# Autodesk Inventor assembly: Ensamblaje carcasa control
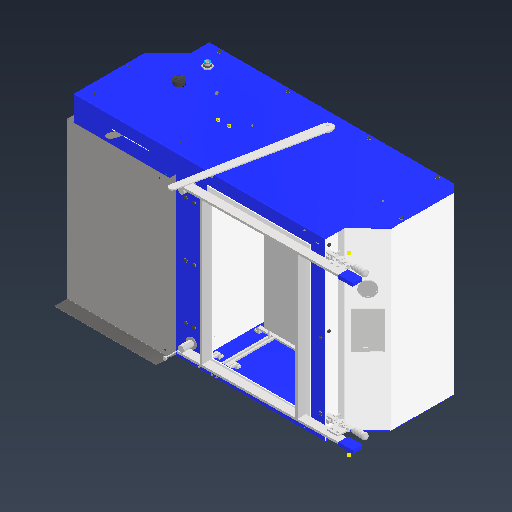
[picture p0: Inventor's stored thumbnail of the model, 512x512]
Saved by Autodesk Inventor 2021 (Build 250183000, 183)
## iProperties
Created: 2021-04-15
Part Number: Ensamblaje carcasa control
Document SubType Name: Assembly
Designer: Admin
Author: Admin
## Documents named in this file (40)
- J:\PAI\Proyecto_PAI_2021\01 CAD\Ensamblaje carcasa control.iam
- J:\PAI\Proyecto_PAI_2021\01 CAD\Carcasa_azul.ipt
- J:\PAI\Proyecto_PAI_2021\01 CAD\Carcaza_blanca_frontal.ipt
- J:\PAI\Proyecto_PAI_2021\01 CAD\Tapa_blanca_inferior.ipt
- J:\PAI\Proyecto_PAI_2021\01 CAD\Vacuometro.ipt
- J:\PAI\Proyecto_PAI_2021\01 CAD\HMI_NV3W_MR20L_V1.iam
- J:\PAI\Proyecto_PAI_2021\01 CAD\Receptaculo e interruptor.ipt
- J:\PAI\Proyecto_PAI_2021\01 CAD\Portafusible para fusible de 13A.ipt
- J:\PAI\Proyecto_PAI_2021\01 CAD\Tapa_interior_1.ipt
- J:\PAI\Proyecto_PAI_2021\01 CAD\Tapa_interior_2.ipt
- J:\PAI\Proyecto_PAI_2021\01 CAD\Tapa_blanca_trasera.ipt
- J:\PAI\Proyecto_PAI_2021\01 CAD\Bomba de Vacio.ipt
- J:\PAI\Proyecto_PAI_2021\01 CAD\Marco molde.ipt
- J:\PAI\Proyecto_PAI_2021\01 CAD\CSN 02 1721 - 17,5.ipt
- J:\PAI\Proyecto_PAI_2021\01 CAD\Ensamblaje_soportme molde_barras.iam
- J:\PAI\Proyecto_PAI_2021\01 CAD\Mecanismo Modelado.iam
- J:\PAI\Proyecto_PAI_2021\01 CAD\Bandeja_proteccion_carcasa_control.ipt
- J:\PAI\Proyecto_PAI_2021\01 CAD\BS 4320 - M5 (Forma A).ipt
- J:\PAI\Proyecto_PAI_2021\01 CAD\ISO 7380-1 - M5 x 8.ipt
- J:\PAI\Proyecto_PAI_2021\01 CAD\BS 4183 - M5(1).ipt
- J:\PAI\Proyecto_PAI_2021\01 CAD\MecanismoBoqueoCarro\ProtectorBloqueo.ipt
- J:\PAI\Proyecto_PAI_2021\01 CAD\Ensamble eléctrico.iam
- J:\PAI\Proyecto_PAI_2021\01 CAD\ISO 7049 - ST 3,5 x 9,5 - C - H.ipt
- J:\PAI\Proyecto_PAI_2021\01 CAD\020sa24.iam
- J:\PAI\Proyecto_PAI_2021\01 CAD\ls-s02-zb.iam
- J:\PAI\Proyecto_PAI_2021\01 CAD\Racor bomba.ipt
- J:\PAI\Proyecto_PAI_2021\01 CAD\2021 C-1_8-P-6.ipt
- J:\PAI\Proyecto_PAI_2021\01 CAD\153160 QSS-10.iam
- J:\PAI\Proyecto_PAI_2021\01 CAD\15631 N-1_4-P-6-MS.ipt
- J:\PAI\Proyecto_PAI_2021\01 CAD\Filtro.iam
- J:\PAI\Proyecto_PAI_2021\01 CAD\Base vacuometro.ipt
- J:\PAI\Proyecto_PAI_2021\01 CAD\BS 4168 - M4 x 20(1).ipt
- J:\PAI\Proyecto_PAI_2021\01 CAD\AS 1112 - M4(2).ipt
- C:\Users\GABRIEL LOL\Desktop\planos pai\mecanismobloq2\MecanismoBloq2.iam
- C:\Users\GABRIEL LOL\Desktop\planos pai\PieDeBomba.iam
- C:\Users\GABRIEL LOL\Documents\Inventor\Content Center Files\R2021\en-US\ISO 7380-1\ISO 7380-1 - M6 x 16.ipt
- C:\Users\GABRIEL LOL\Documents\Inventor\Content Center Files\R2021\en-US\ISO 7092\ISO 7092 - ST 2.5 - 140 HV.ipt
- C:\Users\GABRIEL LOL\Documents\Inventor\Content Center Files\R2021\en-US\ISO 4762(2)\ISO 4762 - M2.5 x 10ISO.ipt
- C:\Users\GABRIEL LOL\Documents\Inventor\Content Center Files\R2021\en-US\ISO 4032(2)\ISO 4032 - M2.5 - ISO.ipt
- C:\Users\GABRIEL LOL\Documents\Inventor\Content Center Files\R2021\en-US\ISO 4762(2)\ISO 4762 - M2.5 x 8ISO.ipt
## Components (183 placed, 39 different names)
1. Carcasa_azul:1 — Coincidencia:1, Nivelación:1, Coincidencia:2, Coincidencia:3, Nivelación:2, Coincidencia:5, Coincidencia:6, Coincidencia:7, Coincidencia:8, Coincidencia:9, Coincidencia:18, Coincidencia:20, Coincidencia:27, Nivelación:6, Nivelación:7, Coincidencia:28, Coincidencia:29, Coincidencia:30, Coincidencia:31, Coincidencia:32, Coincidencia:34, Nivelación:8, Nivelación:9, Coincidencia:35, De rotación:1, De rotación:2, De rotación:4, De rotación:5, De rotación:6, De rotación:7, De rotación:8, De rotación:9, De rotación:10, De rotación:11, De rotación:42, De rotación:48, De rotación:64, De rotación:65, De rotación:66, Coincidencia:36, Mate:38, Coincidencia:39, De rotación:107, De rotación:108, De rotación:109, De rotación:110, De rotación:111, De rotación:112, De rotación:117, Mate:40, Mate:41, Mate:42, Coincidencia:45, Coincidencia:46, De rotación:118, De rotación:119, De rotación:120, De rotación:121, De rotación:122, De rotación:123, Mate:71, Mate:72, Mate:80, Mate:102, Mate:103, Mate:104, Mate:106, Mate:107, Mate:108, Mate:110, Mate:111, Mate:112, Mate:114, Mate:115, Mate:116, Mate:118, Mate:119, Mate:120, Mate:122, Mate:123, Mate:124, Mate:126, Mate:127, Mate:128, Mate:129, Mate:130, Mate:132, Mate:134, Mate:135, Mate:136, Mate:138, Mate:139, Mate:140, Mate:141, Mate:142, Mate:144
2. Carcaza_blanca_frontal:1 — Coincidencia:1, Nivelación:1, Coincidencia:2, Coincidencia:4, Coincidencia:10, Coincidencia:11, Coincidencia:12, Coincidencia:13, Coincidencia:14, Coincidencia:19, De rotación:24, De rotación:25, De rotación:26, De rotación:56, De rotación:57, De rotación:58, Coincidencia:77
3. Tapa_blanca_inferior:1 — Coincidencia:3, Coincidencia:4, Nivelación:2, Nivelación:4, Coincidencia:21, De rotación:38, De rotación:39, De rotación:40, De rotación:41, De rotación:44, De rotación:45, De rotación:46, De rotación:49, De rotación:50, De rotación:51, De rotación:52, De rotación:98, De rotación:99, De rotación:100, De rotación:124, De rotación:125, De rotación:126, De rotación:127, De rotación:128, De rotación:129, Mate:49, Mate:81, Mate:82, Mate:83, Mate:84, Mate:85, Mate:86, Mate:87, Mate:88, Mate:101, Insert:1, Insert:2, Insert:3, Insert:4
4. Vacuometro:1 — Coincidencia:10, Coincidencia:11, Mate:69, Mate:70, Coincidencia:78, Coincidencia:79, De rotación:142, De rotación:143
5. HMI_NV3W_MR20L_V1:1 [sub-assembly] — Coincidencia:12, Coincidencia:13, Coincidencia:14
6. Receptaculo e interruptor:1 — Coincidencia:7, Coincidencia:8, Coincidencia:9
7. Portafusible para fusible de 13A:1 — Coincidencia:5, Coincidencia:6
8. Tapa_interior_2:1 — Coincidencia:18, Coincidencia:19, De rotación:62, De rotación:63, Rígido:1, Coincidencia:44
9. Tapa_blanca_trasera:1 — Coincidencia:20, Nivelación:4, Coincidencia:21, De rotación:104, De rotación:105, De rotación:106
10. Marco molde:1 — Coincidencia:27, Nivelación:6, Nivelación:7
11. CSN 02 1721 17,5:1 — Coincidencia:28, Coincidencia:30, Cilíndrica:1
12. CSN 02 1721 17,5:2 — Coincidencia:29, Coincidencia:31
13. Ensamblaje_soportme molde_barras:1 [sub-assembly] — Cilíndrica:1
14. Mecanismo Modelado:1 [sub-assembly] — Coincidencia:32, Coincidencia:34, Coincidencia:36, Mate:37, Mate:105, Mate:109, Mate:113, Mate:117, Mate:121, Mate:125, Mate:131, Mate:133, Mate:137, Mate:143, Mate:145
15. Bandeja_proteccion_carcasa_control:1 — Nivelación:8, Nivelación:9, Coincidencia:35
16. BS 4320 Forma AB M5 (Forma A):4 — De rotación:1, De rotación:16
17. BS 4320 Forma AB M5 (Forma A):5 — De rotación:2, De rotación:15
18. BS 4320 Forma AB M5 (Forma A):7 — De rotación:4, De rotación:14
19. BS 4320 Forma AB M5 (Forma A):8 — De rotación:5, De rotación:17
20. BS 4320 Forma AB M5 (Forma A):9 — De rotación:6, De rotación:13
21. BS 4320 Forma AB M5 (Forma A):10 — De rotación:9, De rotación:21
22. BS 4320 Forma AB M5 (Forma A):11 — De rotación:7, De rotación:23
23. BS 4320 Forma AB M5 (Forma A):12 — De rotación:11, De rotación:19
24. BS 4320 Forma AB M5 (Forma A):13 — De rotación:8, De rotación:22
25. BS 4320 Forma AB M5 (Forma A):14 — De rotación:10, De rotación:20
26. ISO 7380-1 M5 x 8:1 — De rotación:15
27. ISO 7380-1 M5 x 8:3 — De rotación:17
28. ISO 7380-1 M5 x 8:4 — De rotación:16
29. ISO 7380-1 M5 x 8:5 — De rotación:14
30. ISO 7380-1 M5 x 8:6 — De rotación:13
31. ISO 7380-1 M5 x 8:7 — De rotación:20
32. ISO 7380-1 M5 x 8:8 — De rotación:21
33. ISO 7380-1 M5 x 8:10 — De rotación:23
34. ISO 7380-1 M5 x 8:11 — De rotación:19
35. ISO 7380-1 M5 x 8:12 — De rotación:22
36. ISO 7380-1 M5 x 8:13 — De rotación:27
37. ISO 7380-1 M5 x 8:14 — De rotación:29
38. ISO 7380-1 M5 x 8:15 — De rotación:28
39. BS 4320 Forma AB M5 (Forma A):16 — De rotación:26, De rotación:27
40. BS 4320 Forma AB M5 (Forma A):17 — De rotación:25, De rotación:28
41. BS 4320 Forma AB M5 (Forma A):18 — De rotación:24, De rotación:29
42. BS 4183 - Métrico M5:1 — De rotación:38
43. BS 4183 - Métrico M5:2 — De rotación:39
44. BS 4183 - Métrico M5:3 — De rotación:42
45. BS 4183 - Métrico M5:4 — De rotación:40
46. BS 4183 - Métrico M5:6 — De rotación:41
47. BS 4183 - Métrico M5:7 — De rotación:45
48. BS 4183 - Métrico M5:8 — De rotación:44
49. BS 4183 - Métrico M5:10 — De rotación:46
50. BS 4183 - Métrico M5:11 — De rotación:48
51. BS 4183 - Métrico M5:12 — De rotación:49
52. BS 4183 - Métrico M5:13 — De rotación:50
53. BS 4183 - Métrico M5:14 — De rotación:52
54. BS 4183 - Métrico M5:15 — De rotación:51
55. ISO 7380-1 M5 x 8:21 — De rotación:59
56. ISO 7380-1 M5 x 8:22 — De rotación:60
57. ISO 7380-1 M5 x 8:23 — De rotación:61
58. BS 4320 Forma AB M5 (Forma A):22 — De rotación:57, De rotación:60
59. BS 4320 Forma AB M5 (Forma A):23 — De rotación:58, De rotación:61
60. BS 4320 Forma AB M5 (Forma A):24 — De rotación:56, De rotación:59
61. BS 4183 - Métrico M5:19 — De rotación:62
62. BS 4183 - Métrico M5:20 — De rotación:63
63. BS 4183 - Métrico M5:21 — Rígido:1
64. ISO 7380-1 M5 x 8:24 — De rotación:69
65. ISO 7380-1 M5 x 8:25 — De rotación:68
66. ISO 7380-1 M5 x 8:26 — De rotación:67
67. BS 4320 Forma AB M5 (Forma A):25 — De rotación:66, De rotación:69
68. BS 4320 Forma AB M5 (Forma A):26 — De rotación:65, De rotación:68
69. BS 4320 Forma AB M5 (Forma A):27 — De rotación:64, De rotación:67
70. BS 4183 - Métrico M5:22
71. BS 4183 - Métrico M5:23
72. BS 4183 - Métrico M5:24
73. ProtectorBloqueo:1 — Mate:37, Mate:38
74. Tapa_interior_1:1 — Coincidencia:39, Coincidencia:44, Coincidencia:47
75. Ensamble eléctrico:1 [sub-assembly] — Coincidencia:45, Coincidencia:46, Coincidencia:47, De rotación:146, De rotación:147, De rotación:148, De rotación:149
76. ISO 7380-1 M5 x 8:39 — De rotación:101
77. ISO 7380-1 M5 x 8:40 — De rotación:102
78. ISO 7380-1 M5 x 8:41 — De rotación:103
79. BS 4320 Forma AB M5 (Forma A):40 — De rotación:98, De rotación:101
80. BS 4320 Forma AB M5 (Forma A):41 — De rotación:99, De rotación:102
81. BS 4320 Forma AB M5 (Forma A):42 — De rotación:100, De rotación:103
82. ISO 7049 - C-H ST 3,5 x 9,5 - C - H:1 — De rotación:106
83. ISO 7049 - C-H ST 3,5 x 9,5 - C - H:2 — De rotación:105
84. ISO 7049 - C-H ST 3,5 x 9,5 - C - H:3 — De rotación:104
85. ISO 7049 - C-H ST 3,5 x 9,5 - C - H:4 — De rotación:108
86. ISO 7049 - C-H ST 3,5 x 9,5 - C - H:5 — De rotación:107
87. BS 4320 Forma AB M5 (Forma A):43 — De rotación:112, De rotación:115
88. BS 4320 Forma AB M5 (Forma A):44 — De rotación:111, De rotación:116
89. BS 4320 Forma AB M5 (Forma A):45 — De rotación:110, De rotación:114
90. BS 4320 Forma AB M5 (Forma A):46 — De rotación:109, De rotación:113
91. ISO 7380-1 M5 x 8:42 — De rotación:114
92. ISO 7380-1 M5 x 8:43 — De rotación:113
93. ISO 7380-1 M5 x 8:44 — De rotación:116
94. ISO 7380-1 M5 x 8:45 — De rotación:115
95. BS 4183 - Métrico M5:25 — De rotación:117
96. 020sa24:1 [sub-assembly] — Mate:40, Mate:41
97. ls-s02-zb:1 [sub-assembly] — Mate:42
98. BS 4320 Forma AB M5 (Forma A):47 — De rotación:120, De rotación:133
99. BS 4320 Forma AB M5 (Forma A):48 — De rotación:123, De rotación:130
100. BS 4320 Forma AB M5 (Forma A):49 — De rotación:121, De rotación:132
101. BS 4320 Forma AB M5 (Forma A):50 — De rotación:122, De rotación:131
102. BS 4320 Forma AB M5 (Forma A):51 — De rotación:119, De rotación:134
103. BS 4320 Forma AB M5 (Forma A):52 — De rotación:118, De rotación:135
104. BS 4320 Forma AB M5 (Forma A):53 — De rotación:125, De rotación:141
105. BS 4320 Forma AB M5 (Forma A):54 — De rotación:127, De rotación:139
106. BS 4320 Forma AB M5 (Forma A):55 — De rotación:128, De rotación:136
107. BS 4320 Forma AB M5 (Forma A):56 — De rotación:129, De rotación:137
108. BS 4320 Forma AB M5 (Forma A):57 — De rotación:126, De rotación:138
109. BS 4320 Forma AB M5 (Forma A):58 — De rotación:124, De rotación:140
110. ISO 7380-1 M5 x 8:46 — De rotación:130
111. ISO 7380-1 M5 x 8:47 — De rotación:132
112. ISO 7380-1 M5 x 8:48 — De rotación:135
113. ISO 7380-1 M5 x 8:49 — De rotación:134
114. ISO 7380-1 M5 x 8:50 — De rotación:131
115. ISO 7380-1 M5 x 8:51 — De rotación:133
116. ISO 7380-1 M5 x 8:52 — De rotación:136
117. ISO 7380-1 M5 x 8:53 — De rotación:137
118. ISO 7380-1 M5 x 8:54 — De rotación:138
119. ISO 7380-1 M5 x 8:55 — De rotación:139
120. ISO 7380-1 M5 x 8:56 — De rotación:141
121. ISO 7380-1 M5 x 8:57 — De rotación:140
122. Bomba de Vacio:1 — Mate:49, Mate:50, Mate:51, Mate:52, Mate:53, Mate:89, Mate:90, Mate:91, Mate:92, Mate:93, Mate:94, Mate:95, Mate:96, Mate:97, Mate:98, Mate:99
123. Racor bomba:1 — Mate:50, Mate:51
124. Racor bomba:2 — Mate:52, Mate:53
125. Racor bomba:3 — De rotación:146
126. Racor bomba:4 — De rotación:147
127. Racor bomba:5 — De rotación:149
128. 2021 C-1_8-P-6:1 — Mate:69, Mate:70
129. 153160 QSS-10:1 [sub-assembly] — Mate:71, Mate:72
130. 15631 N-1_4-P-6-MS:2 — De rotación:148
131. Filtro:1 [sub-assembly]
132. Base vacuometro:1 — Coincidencia:77, Coincidencia:78, Coincidencia:79, De rotación:144, De rotación:145
133. BS 4168 : Pieza 1 Tornillo de cabeza cilíndrica con hueco hexagonal - Métrico M4 x 20:1 — De rotación:143
134. BS 4168 : Pieza 1 Tornillo de cabeza cilíndrica con hueco hexagonal - Métrico M4 x 20:2 — De rotación:142
135. AS 1112 (4) - Métrico M4:1 — De rotación:144
136. AS 1112 (4) - Métrico M4:2 — De rotación:145
137. MecanismoBloq2:1 [sub-assembly] — Mate:80
138. PieDeBomba:1 [sub-assembly] — Mate:81, Mate:85, Mate:89, Mate:91, Mate:100
139. PieDeBomba:2 [sub-assembly] — Mate:84, Mate:87
140. PieDeBomba:3 [sub-assembly] — Mate:83, Mate:88, Mate:90
141. PieDeBomba:4 [sub-assembly] — Mate:82, Mate:86
142. ISO 7380-1 M6 x 16:1 — Mate:92, Mate:93
143. ISO 7380-1 M6 x 16:2 — Mate:94, Mate:95
144. ISO 7380-1 M6 x 16:3 — Mate:96, Mate:97
145. ISO 7380-1 M6 x 16:4 — Mate:98, Mate:99
146. ISO 7380-1 M6 x 16:5 — Mate:100, Mate:101
147. ISO 7380-1 M6 x 16:6 — Insert:1
148. ISO 7380-1 M6 x 16:7 — Insert:2
149. ISO 7380-1 M6 x 16:8 — Insert:3
150. ISO 7380-1 M6 x 16:9 — Insert:4
151. ISO 7092 ST 2.5 - 140 HV:1 — Mate:102, Mate:103, Insert:5
152. ISO 4762 M2.5 x 10:1 — Insert:5
153. ISO 4032 M2.5:1 — Mate:104, Mate:105
154. ISO 7092 ST 2.5 - 140 HV:2 — Mate:106, Mate:107, Insert:6
155. ISO 4762 M2.5 x 10:2 — Insert:6
156. ISO 4032 M2.5:2 — Mate:108, Mate:109
157. ISO 7092 ST 2.5 - 140 HV:3 — Mate:110, Mate:111, Insert:7
158. ISO 4762 M2.5 x 10:3 — Insert:7
159. ISO 4032 M2.5:3 — Mate:112, Mate:113
160. ISO 7092 ST 2.5 - 140 HV:4 — Mate:114, Mate:115, Insert:8
161. ISO 4762 M2.5 x 10:4 — Insert:8
162. ISO 4032 M2.5:4 — Mate:116, Mate:117
163. ISO 7092 ST 2.5 - 140 HV:5 — Mate:118, Mate:119, Insert:9
164. ISO 4762 M2.5 x 10:5 — Insert:9
165. ISO 4032 M2.5:5 — Mate:120, Mate:121
166. ISO 7092 ST 2.5 - 140 HV:6 — Mate:122, Mate:123, Insert:10
167. ISO 4762 M2.5 x 10:6 — Insert:10
168. ISO 4032 M2.5:6 — Mate:124, Mate:125
169. ISO 7092 ST 2.5 - 140 HV:7 — Mate:126, Mate:127, Insert:11
170. ISO 4762 M2.5 x 8:1 — Insert:11
171. ISO 4032 M2.5:7 — Mate:130, Mate:131
172. ISO 7092 ST 2.5 - 140 HV:8 — Mate:128, Mate:129, Insert:12
173. ISO 4762 M2.5 x 8:2 — Insert:12
174. ISO 4032 M2.5:8 — Mate:132, Mate:133
175. ISO 7092 ST 2.5 - 140 HV:9 — Mate:134, Mate:135, Insert:13
176. ISO 4762 M2.5 x 10:7 — Insert:13
177. ISO 4032 M2.5:9 — Mate:136, Mate:137
178. ISO 7092 ST 2.5 - 140 HV:10 — Mate:138, Mate:139, Insert:14
179. ISO 4762 M2.5 x 10:8 — Insert:14
180. ISO 4032 M2.5:10 — Mate:142, Mate:143
181. ISO 7092 ST 2.5 - 140 HV:11 — Mate:140, Mate:141, Insert:15
182. ISO 4762 M2.5 x 10:9 — Insert:15
183. ISO 4032 M2.5:11 — Mate:144, Mate:145
## Relationships (244: Mate 115, RevoluteJoint 105, Insert 15, Flush 7, CylindricalJoint 1, WeldJoint 1)
- Coincidencia:1 [Mate]: Carcasa_azul:1 ↔ Carcaza_blanca_frontal:1
- Nivelación:1 [Flush]: Carcasa_azul:1 ↔ Carcaza_blanca_frontal:1
- Coincidencia:2 [Mate]: Carcasa_azul:1 ↔ Carcaza_blanca_frontal:1
- Coincidencia:3 [Mate]: Carcasa_azul:1 ↔ Tapa_blanca_inferior:1
- Coincidencia:4 [Mate]: Carcaza_blanca_frontal:1 ↔ Tapa_blanca_inferior:1
- Nivelación:2 [Flush]: Carcasa_azul:1 ↔ Tapa_blanca_inferior:1
- Coincidencia:5 [Mate]: Carcasa_azul:1 ↔ Portafusible para fusible de 13A:1
- Coincidencia:6 [Mate]: Carcasa_azul:1 ↔ Portafusible para fusible de 13A:1
- Coincidencia:7 [Mate]: Carcasa_azul:1 ↔ Receptaculo e interruptor:1
- Coincidencia:8 [Mate]: Carcasa_azul:1 ↔ Receptaculo e interruptor:1
- Coincidencia:9 [Mate]: Carcasa_azul:1 ↔ Receptaculo e interruptor:1
- Coincidencia:10 [Mate]: Carcaza_blanca_frontal:1 ↔ Vacuometro:1
- Coincidencia:11 [Mate]: Carcaza_blanca_frontal:1 ↔ Vacuometro:1
- Coincidencia:12 [Mate]: Carcaza_blanca_frontal:1 ↔ HMI_NV3W_MR20L_V1:1
- Coincidencia:13 [Mate]: Carcaza_blanca_frontal:1 ↔ HMI_NV3W_MR20L_V1:1
- Coincidencia:14 [Mate]: Carcaza_blanca_frontal:1 ↔ HMI_NV3W_MR20L_V1:1
- Coincidencia:18 [Mate]: Carcasa_azul:1 ↔ Tapa_interior_2:1
- Coincidencia:19 [Mate]: Carcaza_blanca_frontal:1 ↔ Tapa_interior_2:1
- Coincidencia:20 [Mate]: Carcasa_azul:1 ↔ Tapa_blanca_trasera:1
- Nivelación:4 [Flush]: Tapa_blanca_inferior:1 ↔ Tapa_blanca_trasera:1
- Coincidencia:21 [Mate]: Tapa_blanca_inferior:1 ↔ Tapa_blanca_trasera:1
- Coincidencia:27 [Mate]: Carcasa_azul:1 ↔ Marco molde:1
- Nivelación:6 [Flush]: Carcasa_azul:1 ↔ Marco molde:1
- Nivelación:7 [Flush]: Carcasa_azul:1 ↔ Marco molde:1
- Coincidencia:28 [Mate]: Carcasa_azul:1 ↔ CSN 02 1721 17,5:1
- Coincidencia:29 [Mate]: Carcasa_azul:1 ↔ CSN 02 1721 17,5:2
- Coincidencia:30 [Mate]: Carcasa_azul:1 ↔ CSN 02 1721 17,5:1
- Coincidencia:31 [Mate]: Carcasa_azul:1 ↔ CSN 02 1721 17,5:2
- Cilíndrica:1 [CylindricalJoint]: CSN 02 1721 17,5:1 ↔ Ensamblaje_soportme molde_barras:1
- Coincidencia:32 [Mate]: Carcasa_azul:1 ↔ Mecanismo Modelado:1
- Coincidencia:34 [Mate]: Carcasa_azul:1 ↔ Mecanismo Modelado:1
- Nivelación:8 [Flush] (5 mm): Carcasa_azul:1 ↔ Bandeja_proteccion_carcasa_control:1
- Nivelación:9 [Flush]: Carcasa_azul:1 ↔ Bandeja_proteccion_carcasa_control:1
- Coincidencia:35 [Mate]: Carcasa_azul:1 ↔ Bandeja_proteccion_carcasa_control:1
- De rotación:1 [RevoluteJoint]: Carcasa_azul:1 ↔ BS 4320 Forma AB M5 (Forma A):4
- De rotación:2 [RevoluteJoint]: Carcasa_azul:1 ↔ BS 4320 Forma AB M5 (Forma A):5
- De rotación:4 [RevoluteJoint]: Carcasa_azul:1 ↔ BS 4320 Forma AB M5 (Forma A):7
- De rotación:5 [RevoluteJoint]: Carcasa_azul:1 ↔ BS 4320 Forma AB M5 (Forma A):8
- De rotación:6 [RevoluteJoint]: Carcasa_azul:1 ↔ BS 4320 Forma AB M5 (Forma A):9
- De rotación:7 [RevoluteJoint]: Carcasa_azul:1 ↔ BS 4320 Forma AB M5 (Forma A):11
- De rotación:8 [RevoluteJoint]: Carcasa_azul:1 ↔ BS 4320 Forma AB M5 (Forma A):13
- De rotación:9 [RevoluteJoint]: Carcasa_azul:1 ↔ BS 4320 Forma AB M5 (Forma A):10
- De rotación:10 [RevoluteJoint]: Carcasa_azul:1 ↔ BS 4320 Forma AB M5 (Forma A):14
- De rotación:11 [RevoluteJoint]: Carcasa_azul:1 ↔ BS 4320 Forma AB M5 (Forma A):12
- De rotación:13 [RevoluteJoint]: BS 4320 Forma AB M5 (Forma A):9 ↔ ISO 7380-1 M5 x 8:6
- De rotación:14 [RevoluteJoint]: BS 4320 Forma AB M5 (Forma A):7 ↔ ISO 7380-1 M5 x 8:5
- De rotación:15 [RevoluteJoint]: BS 4320 Forma AB M5 (Forma A):5 ↔ ISO 7380-1 M5 x 8:1
- De rotación:16 [RevoluteJoint]: BS 4320 Forma AB M5 (Forma A):4 ↔ ISO 7380-1 M5 x 8:4
- De rotación:17 [RevoluteJoint]: BS 4320 Forma AB M5 (Forma A):8 ↔ ISO 7380-1 M5 x 8:3
- De rotación:19 [RevoluteJoint]: BS 4320 Forma AB M5 (Forma A):12 ↔ ISO 7380-1 M5 x 8:11
- De rotación:20 [RevoluteJoint]: BS 4320 Forma AB M5 (Forma A):14 ↔ ISO 7380-1 M5 x 8:7
- De rotación:21 [RevoluteJoint]: BS 4320 Forma AB M5 (Forma A):10 ↔ ISO 7380-1 M5 x 8:8
- De rotación:22 [RevoluteJoint]: BS 4320 Forma AB M5 (Forma A):13 ↔ ISO 7380-1 M5 x 8:12
- De rotación:23 [RevoluteJoint]: BS 4320 Forma AB M5 (Forma A):11 ↔ ISO 7380-1 M5 x 8:10
- De rotación:24 [RevoluteJoint]: Carcaza_blanca_frontal:1 ↔ BS 4320 Forma AB M5 (Forma A):18
- De rotación:25 [RevoluteJoint]: Carcaza_blanca_frontal:1 ↔ BS 4320 Forma AB M5 (Forma A):17
- De rotación:26 [RevoluteJoint]: Carcaza_blanca_frontal:1 ↔ BS 4320 Forma AB M5 (Forma A):16
- De rotación:27 [RevoluteJoint]: ISO 7380-1 M5 x 8:13 ↔ BS 4320 Forma AB M5 (Forma A):16
- De rotación:28 [RevoluteJoint]: ISO 7380-1 M5 x 8:15 ↔ BS 4320 Forma AB M5 (Forma A):17
- De rotación:29 [RevoluteJoint]: ISO 7380-1 M5 x 8:14 ↔ BS 4320 Forma AB M5 (Forma A):18
- De rotación:38 [RevoluteJoint]: Tapa_blanca_inferior:1 ↔ BS 4183 - Métrico M5:1
- De rotación:39 [RevoluteJoint]: Tapa_blanca_inferior:1 ↔ BS 4183 - Métrico M5:2
- De rotación:40 [RevoluteJoint]: Tapa_blanca_inferior:1 ↔ BS 4183 - Métrico M5:4
- De rotación:41 [RevoluteJoint]: Tapa_blanca_inferior:1 ↔ BS 4183 - Métrico M5:6
- De rotación:42 [RevoluteJoint]: Carcasa_azul:1 ↔ BS 4183 - Métrico M5:3
- De rotación:44 [RevoluteJoint]: Tapa_blanca_inferior:1 ↔ BS 4183 - Métrico M5:8
- De rotación:45 [RevoluteJoint]: Tapa_blanca_inferior:1 ↔ BS 4183 - Métrico M5:7
- De rotación:46 [RevoluteJoint]: Tapa_blanca_inferior:1 ↔ BS 4183 - Métrico M5:10
- De rotación:48 [RevoluteJoint]: Carcasa_azul:1 ↔ BS 4183 - Métrico M5:11
- De rotación:49 [RevoluteJoint]: Tapa_blanca_inferior:1 ↔ BS 4183 - Métrico M5:12
- De rotación:50 [RevoluteJoint]: Tapa_blanca_inferior:1 ↔ BS 4183 - Métrico M5:13
- De rotación:51 [RevoluteJoint]: Tapa_blanca_inferior:1 ↔ BS 4183 - Métrico M5:15
- De rotación:52 [RevoluteJoint]: Tapa_blanca_inferior:1 ↔ BS 4183 - Métrico M5:14
- De rotación:56 [RevoluteJoint]: Carcaza_blanca_frontal:1 ↔ BS 4320 Forma AB M5 (Forma A):24
- De rotación:57 [RevoluteJoint]: Carcaza_blanca_frontal:1 ↔ BS 4320 Forma AB M5 (Forma A):22
- De rotación:58 [RevoluteJoint]: Carcaza_blanca_frontal:1 ↔ BS 4320 Forma AB M5 (Forma A):23
- De rotación:59 [RevoluteJoint]: ISO 7380-1 M5 x 8:21 ↔ BS 4320 Forma AB M5 (Forma A):24
- De rotación:60 [RevoluteJoint]: ISO 7380-1 M5 x 8:22 ↔ BS 4320 Forma AB M5 (Forma A):22
- De rotación:61 [RevoluteJoint]: ISO 7380-1 M5 x 8:23 ↔ BS 4320 Forma AB M5 (Forma A):23
- De rotación:62 [RevoluteJoint]: Tapa_interior_2:1 ↔ BS 4183 - Métrico M5:19
- De rotación:63 [RevoluteJoint]: Tapa_interior_2:1 ↔ BS 4183 - Métrico M5:20
- Rígido:1 [WeldJoint]: Tapa_interior_2:1 ↔ BS 4183 - Métrico M5:21
- De rotación:64 [RevoluteJoint]: Carcasa_azul:1 ↔ BS 4320 Forma AB M5 (Forma A):27
- De rotación:65 [RevoluteJoint]: Carcasa_azul:1 ↔ BS 4320 Forma AB M5 (Forma A):26
- De rotación:66 [RevoluteJoint]: Carcasa_azul:1 ↔ BS 4320 Forma AB M5 (Forma A):25
- De rotación:67 [RevoluteJoint]: ISO 7380-1 M5 x 8:26 ↔ BS 4320 Forma AB M5 (Forma A):27
- De rotación:68 [RevoluteJoint]: ISO 7380-1 M5 x 8:25 ↔ BS 4320 Forma AB M5 (Forma A):26
- De rotación:69 [RevoluteJoint]: ISO 7380-1 M5 x 8:24 ↔ BS 4320 Forma AB M5 (Forma A):25
- Coincidencia:36 [Mate]: Carcasa_azul:1 ↔ Mecanismo Modelado:1
- Mate:37: Mecanismo Modelado:1 ↔ ProtectorBloqueo:1
- Mate:38: Carcasa_azul:1 ↔ ProtectorBloqueo:1
- Coincidencia:39 [Mate]: Carcasa_azul:1 ↔ Tapa_interior_1:1
- De rotación:98 [RevoluteJoint]: Tapa_blanca_inferior:1 ↔ BS 4320 Forma AB M5 (Forma A):40
- De rotación:99 [RevoluteJoint]: Tapa_blanca_inferior:1 ↔ BS 4320 Forma AB M5 (Forma A):41
- De rotación:100 [RevoluteJoint]: Tapa_blanca_inferior:1 ↔ BS 4320 Forma AB M5 (Forma A):42
- De rotación:101 [RevoluteJoint]: ISO 7380-1 M5 x 8:39 ↔ BS 4320 Forma AB M5 (Forma A):40
- De rotación:102 [RevoluteJoint]: ISO 7380-1 M5 x 8:40 ↔ BS 4320 Forma AB M5 (Forma A):41
- De rotación:103 [RevoluteJoint]: ISO 7380-1 M5 x 8:41 ↔ BS 4320 Forma AB M5 (Forma A):42
- De rotación:104 [RevoluteJoint]: Tapa_blanca_trasera:1 ↔ ISO 7049 - C-H ST 3,5 x 9,5 - C - H:3
- De rotación:105 [RevoluteJoint]: Tapa_blanca_trasera:1 ↔ ISO 7049 - C-H ST 3,5 x 9,5 - C - H:2
- De rotación:106 [RevoluteJoint]: Tapa_blanca_trasera:1 ↔ ISO 7049 - C-H ST 3,5 x 9,5 - C - H:1
- De rotación:107 [RevoluteJoint]: Carcasa_azul:1 ↔ ISO 7049 - C-H ST 3,5 x 9,5 - C - H:5
- De rotación:108 [RevoluteJoint]: Carcasa_azul:1 ↔ ISO 7049 - C-H ST 3,5 x 9,5 - C - H:4
- De rotación:109 [RevoluteJoint]: Carcasa_azul:1 ↔ BS 4320 Forma AB M5 (Forma A):46
- De rotación:110 [RevoluteJoint]: Carcasa_azul:1 ↔ BS 4320 Forma AB M5 (Forma A):45
- De rotación:111 [RevoluteJoint]: Carcasa_azul:1 ↔ BS 4320 Forma AB M5 (Forma A):44
- De rotación:112 [RevoluteJoint]: Carcasa_azul:1 ↔ BS 4320 Forma AB M5 (Forma A):43
- De rotación:113 [RevoluteJoint]: BS 4320 Forma AB M5 (Forma A):46 ↔ ISO 7380-1 M5 x 8:43
- De rotación:114 [RevoluteJoint]: BS 4320 Forma AB M5 (Forma A):45 ↔ ISO 7380-1 M5 x 8:42
- De rotación:115 [RevoluteJoint]: BS 4320 Forma AB M5 (Forma A):43 ↔ ISO 7380-1 M5 x 8:45
- De rotación:116 [RevoluteJoint]: BS 4320 Forma AB M5 (Forma A):44 ↔ ISO 7380-1 M5 x 8:44
- De rotación:117 [RevoluteJoint]: Carcasa_azul:1 ↔ BS 4183 - Métrico M5:25
- Mate:40: Carcasa_azul:1 ↔ 020sa24:1
- Mate:41: Carcasa_azul:1 ↔ 020sa24:1
- Mate:42: Carcasa_azul:1 ↔ ls-s02-zb:1
- Coincidencia:44 [Mate] (360 mm): Tapa_interior_2:1 ↔ Tapa_interior_1:1
- Coincidencia:45 [Mate]: Carcasa_azul:1 ↔ Ensamble eléctrico:1
- Coincidencia:46 [Mate] (23.79 mm): Carcasa_azul:1 ↔ Ensamble eléctrico:1
- Coincidencia:47 [Mate] (50 mm): Tapa_interior_1:1 ↔ Ensamble eléctrico:1
- De rotación:118 [RevoluteJoint]: Carcasa_azul:1 ↔ BS 4320 Forma AB M5 (Forma A):52
- De rotación:119 [RevoluteJoint]: Carcasa_azul:1 ↔ BS 4320 Forma AB M5 (Forma A):51
- De rotación:120 [RevoluteJoint]: Carcasa_azul:1 ↔ BS 4320 Forma AB M5 (Forma A):47
- De rotación:121 [RevoluteJoint]: Carcasa_azul:1 ↔ BS 4320 Forma AB M5 (Forma A):49
- De rotación:122 [RevoluteJoint]: Carcasa_azul:1 ↔ BS 4320 Forma AB M5 (Forma A):50
- De rotación:123 [RevoluteJoint]: Carcasa_azul:1 ↔ BS 4320 Forma AB M5 (Forma A):48
- De rotación:124 [RevoluteJoint]: Tapa_blanca_inferior:1 ↔ BS 4320 Forma AB M5 (Forma A):58
- De rotación:125 [RevoluteJoint]: Tapa_blanca_inferior:1 ↔ BS 4320 Forma AB M5 (Forma A):53
- De rotación:126 [RevoluteJoint]: Tapa_blanca_inferior:1 ↔ BS 4320 Forma AB M5 (Forma A):57
- De rotación:127 [RevoluteJoint]: Tapa_blanca_inferior:1 ↔ BS 4320 Forma AB M5 (Forma A):54
- De rotación:128 [RevoluteJoint]: Tapa_blanca_inferior:1 ↔ BS 4320 Forma AB M5 (Forma A):55
- De rotación:129 [RevoluteJoint]: Tapa_blanca_inferior:1 ↔ BS 4320 Forma AB M5 (Forma A):56
- De rotación:130 [RevoluteJoint]: BS 4320 Forma AB M5 (Forma A):48 ↔ ISO 7380-1 M5 x 8:46
- De rotación:131 [RevoluteJoint]: BS 4320 Forma AB M5 (Forma A):50 ↔ ISO 7380-1 M5 x 8:50
- De rotación:132 [RevoluteJoint]: BS 4320 Forma AB M5 (Forma A):49 ↔ ISO 7380-1 M5 x 8:47
- De rotación:133 [RevoluteJoint]: BS 4320 Forma AB M5 (Forma A):47 ↔ ISO 7380-1 M5 x 8:51
- De rotación:134 [RevoluteJoint]: BS 4320 Forma AB M5 (Forma A):51 ↔ ISO 7380-1 M5 x 8:49
- De rotación:135 [RevoluteJoint]: BS 4320 Forma AB M5 (Forma A):52 ↔ ISO 7380-1 M5 x 8:48
- De rotación:136 [RevoluteJoint]: BS 4320 Forma AB M5 (Forma A):55 ↔ ISO 7380-1 M5 x 8:52
- De rotación:137 [RevoluteJoint]: BS 4320 Forma AB M5 (Forma A):56 ↔ ISO 7380-1 M5 x 8:53
- De rotación:138 [RevoluteJoint]: BS 4320 Forma AB M5 (Forma A):57 ↔ ISO 7380-1 M5 x 8:54
- De rotación:139 [RevoluteJoint]: BS 4320 Forma AB M5 (Forma A):54 ↔ ISO 7380-1 M5 x 8:55
- De rotación:140 [RevoluteJoint]: BS 4320 Forma AB M5 (Forma A):58 ↔ ISO 7380-1 M5 x 8:57
- De rotación:141 [RevoluteJoint]: BS 4320 Forma AB M5 (Forma A):53 ↔ ISO 7380-1 M5 x 8:56
- Mate:49 (90 mm): Tapa_blanca_inferior:1 ↔ Bomba de Vacio:1
- Mate:50: Bomba de Vacio:1 ↔ Racor bomba:1
- Mate:51: Bomba de Vacio:1 ↔ Racor bomba:1
- Mate:52: Bomba de Vacio:1 ↔ Racor bomba:2
- Mate:53: Bomba de Vacio:1 ↔ Racor bomba:2
- Mate:69: Vacuometro:1 ↔ 2021 C-1_8-P-6:1
- Mate:70: Vacuometro:1 ↔ 2021 C-1_8-P-6:1
- Mate:71: Carcasa_azul:1 ↔ 153160 QSS-10:1
- Mate:72: Carcasa_azul:1 ↔ 153160 QSS-10:1
- Coincidencia:77 [Mate]: Carcaza_blanca_frontal:1 ↔ Base vacuometro:1
- Coincidencia:78 [Mate]: Vacuometro:1 ↔ Base vacuometro:1
- Coincidencia:79 [Mate]: Vacuometro:1 ↔ Base vacuometro:1
- De rotación:142 [RevoluteJoint]: Vacuometro:1 ↔ BS 4168 : Pieza 1 Tornillo de cabeza cilíndrica con hueco hexagonal - Métrico M4 x 20:2
- De rotación:143 [RevoluteJoint]: Vacuometro:1 ↔ BS 4168 : Pieza 1 Tornillo de cabeza cilíndrica con hueco hexagonal - Métrico M4 x 20:1
- De rotación:144 [RevoluteJoint]: Base vacuometro:1 ↔ AS 1112 (4) - Métrico M4:1
- De rotación:145 [RevoluteJoint]: Base vacuometro:1 ↔ AS 1112 (4) - Métrico M4:2
- De rotación:146 [RevoluteJoint]: Ensamble eléctrico:1 ↔ Racor bomba:3
- De rotación:147 [RevoluteJoint]: Ensamble eléctrico:1 ↔ Racor bomba:4
- De rotación:148 [RevoluteJoint]: Ensamble eléctrico:1 ↔ 15631 N-1_4-P-6-MS:2
- De rotación:149 [RevoluteJoint]: Ensamble eléctrico:1 ↔ Racor bomba:5
- Mate:80: Carcasa_azul:1 ↔ MecanismoBloq2:1
- Mate:81: Tapa_blanca_inferior:1 ↔ PieDeBomba:1
- Mate:82: Tapa_blanca_inferior:1 ↔ PieDeBomba:4
- Mate:83: Tapa_blanca_inferior:1 ↔ PieDeBomba:3
- Mate:84: Tapa_blanca_inferior:1 ↔ PieDeBomba:2
- Mate:85: Tapa_blanca_inferior:1 ↔ PieDeBomba:1
- Mate:86: Tapa_blanca_inferior:1 ↔ PieDeBomba:4
- Mate:87: Tapa_blanca_inferior:1 ↔ PieDeBomba:2
- Mate:88: Tapa_blanca_inferior:1 ↔ PieDeBomba:3
- Mate:89: Bomba de Vacio:1 ↔ PieDeBomba:1
- Mate:90: Bomba de Vacio:1 ↔ PieDeBomba:3
- Mate:91: Bomba de Vacio:1 ↔ PieDeBomba:1
- Mate:92: Bomba de Vacio:1 ↔ ISO 7380-1 M6 x 16:1
- Mate:93: Bomba de Vacio:1 ↔ ISO 7380-1 M6 x 16:1
- Mate:94: Bomba de Vacio:1 ↔ ISO 7380-1 M6 x 16:2
- Mate:95: Bomba de Vacio:1 ↔ ISO 7380-1 M6 x 16:2
- Mate:96: Bomba de Vacio:1 ↔ ISO 7380-1 M6 x 16:3
- Mate:97: Bomba de Vacio:1 ↔ ISO 7380-1 M6 x 16:3
- Mate:98: Bomba de Vacio:1 ↔ ISO 7380-1 M6 x 16:4
- Mate:99: Bomba de Vacio:1 ↔ ISO 7380-1 M6 x 16:4
- Mate:100: PieDeBomba:1 ↔ ISO 7380-1 M6 x 16:5
- Mate:101: Tapa_blanca_inferior:1 ↔ ISO 7380-1 M6 x 16:5
- Insert:1: Tapa_blanca_inferior:1 ↔ ISO 7380-1 M6 x 16:6
- Insert:2: Tapa_blanca_inferior:1 ↔ ISO 7380-1 M6 x 16:7
- Insert:3: Tapa_blanca_inferior:1 ↔ ISO 7380-1 M6 x 16:8
- Insert:4: Tapa_blanca_inferior:1 ↔ ISO 7380-1 M6 x 16:9
- Mate:102: Carcasa_azul:1 ↔ ISO 7092 ST 2.5 - 140 HV:1
- Mate:103: Carcasa_azul:1 ↔ ISO 7092 ST 2.5 - 140 HV:1
- Insert:5: ISO 7092 ST 2.5 - 140 HV:1 ↔ ISO 4762 M2.5 x 10:1
- Mate:104: Carcasa_azul:1 ↔ ISO 4032 M2.5:1
- Mate:105: Mecanismo Modelado:1 ↔ ISO 4032 M2.5:1
- Mate:106: Carcasa_azul:1 ↔ ISO 7092 ST 2.5 - 140 HV:2
- Mate:107: Carcasa_azul:1 ↔ ISO 7092 ST 2.5 - 140 HV:2
- Insert:6: ISO 7092 ST 2.5 - 140 HV:2 ↔ ISO 4762 M2.5 x 10:2
- Mate:108: Carcasa_azul:1 ↔ ISO 4032 M2.5:2
- Mate:109: Mecanismo Modelado:1 ↔ ISO 4032 M2.5:2
- Mate:110: Carcasa_azul:1 ↔ ISO 7092 ST 2.5 - 140 HV:3
- Mate:111: Carcasa_azul:1 ↔ ISO 7092 ST 2.5 - 140 HV:3
- Insert:7: ISO 7092 ST 2.5 - 140 HV:3 ↔ ISO 4762 M2.5 x 10:3
- Mate:112: Carcasa_azul:1 ↔ ISO 4032 M2.5:3
- Mate:113: Mecanismo Modelado:1 ↔ ISO 4032 M2.5:3
- Mate:114: Carcasa_azul:1 ↔ ISO 7092 ST 2.5 - 140 HV:4
- Mate:115: Carcasa_azul:1 ↔ ISO 7092 ST 2.5 - 140 HV:4
- Insert:8: ISO 7092 ST 2.5 - 140 HV:4 ↔ ISO 4762 M2.5 x 10:4
- Mate:116: Carcasa_azul:1 ↔ ISO 4032 M2.5:4
- Mate:117: Mecanismo Modelado:1 ↔ ISO 4032 M2.5:4
- Mate:118: Carcasa_azul:1 ↔ ISO 7092 ST 2.5 - 140 HV:5
- Mate:119: Carcasa_azul:1 ↔ ISO 7092 ST 2.5 - 140 HV:5
- Insert:9: ISO 7092 ST 2.5 - 140 HV:5 ↔ ISO 4762 M2.5 x 10:5
- Mate:120: Carcasa_azul:1 ↔ ISO 4032 M2.5:5
- Mate:121: Mecanismo Modelado:1 ↔ ISO 4032 M2.5:5
- Mate:122: Carcasa_azul:1 ↔ ISO 7092 ST 2.5 - 140 HV:6
- Mate:123: Carcasa_azul:1 ↔ ISO 7092 ST 2.5 - 140 HV:6
- Insert:10: ISO 7092 ST 2.5 - 140 HV:6 ↔ ISO 4762 M2.5 x 10:6
- Mate:124: Carcasa_azul:1 ↔ ISO 4032 M2.5:6
- Mate:125: Mecanismo Modelado:1 ↔ ISO 4032 M2.5:6
- Mate:126: Carcasa_azul:1 ↔ ISO 7092 ST 2.5 - 140 HV:7
- Mate:127: Carcasa_azul:1 ↔ ISO 7092 ST 2.5 - 140 HV:7
- Mate:128: Carcasa_azul:1 ↔ ISO 7092 ST 2.5 - 140 HV:8
- Mate:129: Carcasa_azul:1 ↔ ISO 7092 ST 2.5 - 140 HV:8
- Insert:11: ISO 7092 ST 2.5 - 140 HV:7 ↔ ISO 4762 M2.5 x 8:1
- Insert:12: ISO 7092 ST 2.5 - 140 HV:8 ↔ ISO 4762 M2.5 x 8:2
- Mate:130: Carcasa_azul:1 ↔ ISO 4032 M2.5:7
- Mate:131: Mecanismo Modelado:1 ↔ ISO 4032 M2.5:7
- Mate:132: Carcasa_azul:1 ↔ ISO 4032 M2.5:8
- Mate:133: Mecanismo Modelado:1 ↔ ISO 4032 M2.5:8
- Mate:134: Carcasa_azul:1 ↔ ISO 7092 ST 2.5 - 140 HV:9
- Mate:135: Carcasa_azul:1 ↔ ISO 7092 ST 2.5 - 140 HV:9
- Insert:13: ISO 7092 ST 2.5 - 140 HV:9 ↔ ISO 4762 M2.5 x 10:7
- Mate:136: Carcasa_azul:1 ↔ ISO 4032 M2.5:9
- Mate:137: Mecanismo Modelado:1 ↔ ISO 4032 M2.5:9
- Mate:138: Carcasa_azul:1 ↔ ISO 7092 ST 2.5 - 140 HV:10
- Mate:139: Carcasa_azul:1 ↔ ISO 7092 ST 2.5 - 140 HV:10
- Mate:140: Carcasa_azul:1 ↔ ISO 7092 ST 2.5 - 140 HV:11
- Mate:141: Carcasa_azul:1 ↔ ISO 7092 ST 2.5 - 140 HV:11
- Insert:14: ISO 7092 ST 2.5 - 140 HV:10 ↔ ISO 4762 M2.5 x 10:8
- Insert:15: ISO 7092 ST 2.5 - 140 HV:11 ↔ ISO 4762 M2.5 x 10:9
- Mate:142: Carcasa_azul:1 ↔ ISO 4032 M2.5:10
- Mate:143: Mecanismo Modelado:1 ↔ ISO 4032 M2.5:10
- Mate:144: Carcasa_azul:1 ↔ ISO 4032 M2.5:11
- Mate:145: Mecanismo Modelado:1 ↔ ISO 4032 M2.5:11
